# Autodesk Inventor assembly: 前後直動
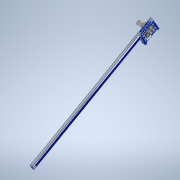
[picture p0: Inventor's stored thumbnail of the model, 180x180]
Saved by Autodesk Inventor 2020.3 (Build 243373000, 373)
## iProperties
Created: 2020-07-05
Part Number: 前後直動
Document SubType Name: Assembly
Designer: totot
Mass: 657.606 g
Surface Area: 2611.22 cm^2
Volume: 274.849 cm^3
Density: 2.39261 g/cm^3
Author: totot
## Documents named in this file (10)
- D:\mysvn\ロボコン\キャチロボ\キャチロボ設計図\ロボット\ハンド\前後直動.iam
- D:\mysvn\ロボコン\キャチロボ\キャチロボ設計図\ロボット\ハンド\12ｘ12_1.ipt
- D:\mysvn\ロボコン\キャチロボ\キャチロボ設計図\ロボット\共有パーツ\DR1-2000_On2.ipt
- D:\mysvn\ロボコン\キャチロボ\キャチロボ設計図\ロボット\ハンド\前後直動12x12_2.ipt
- D:\mysvn\ロボコン\キャチロボ\キャチロボ設計図\ロボット\ハンド\前後直動12x12_3.ipt
- D:\mysvn\ロボコン\キャチロボ\キャチロボ設計図\ロボット\ハンド\前後直動12x12_4.ipt
- D:\mysvn\ロボコン\キャチロボ\キャチロボ設計図\ロボット\共有パーツ\RS_380.ipt
- D:\mysvn\ロボコン\キャチロボ\キャチロボ設計図\ロボット\ハンド\前後直動9x9x24.ipt
- D:\mysvn\ロボコン\キャチロボ\キャチロボ設計図\ロボット\共有パーツ\ポテンションメーター_BI-7284.ipt
- D:\mysvn\ロボコン\キャチロボ\キャチロボ設計図\ロボット\共有パーツ\PS1-20_On.ipt
## Components (14 placed, 9 different names)
1. 12ｘ12_1:1 — メイト:1, フラッシュ:1, フラッシュ:2, 挿入:17, 挿入:18, 挿入:19, 挿入:20, 挿入:21, 挿入:26, 挿入:31, 挿入:32, 挿入:34, 挿入:35
2. DR1-2000_On2:1 — メイト:1, フラッシュ:1, フラッシュ:2
3. 前後直動t5_1 — 挿入:15, 挿入:16, 挿入:20, 挿入:21, 挿入:22, 挿入:23, 正接:1, メイト:2
4. RS_380:1 — 挿入:15, 挿入:16
5. 12ｘ12_1:2 — 挿入:17, 挿入:18, 挿入:19
6. 前後直動12x12_3:1 — 挿入:22, 挿入:23, 挿入:24, 挿入:25, 挿入:27, 挿入:30
7. 前後直動12x12_2:1 — 挿入:24, 挿入:28, 挿入:31, 挿入:36
8. 前後直動12x12_2:2 — 挿入:25, 挿入:26, 挿入:29, 挿入:32, 挿入:33
9. 前後直動9x9x24:1 — 挿入:27, 挿入:29
10. 前後直動9x9x24:2 — 挿入:28, 挿入:30
11. 前後直動9x9x24:3 — 挿入:33, 挿入:34
12. 前後直動9x9x24:4 — 挿入:35, 挿入:36
13. ポテンションメーター_BI-7284:1 — 正接:1, メイト:2, 正接:2, メイト:3
14. PS1-20_On:1 — 正接:2, メイト:3
## Relationships (29: Insert 22, Mate 3, Flush 2, Tangent 2)
- メイト:1 [Mate]: 12ｘ12_1:1 ↔ DR1-2000_On2:1
- フラッシュ:1 [Flush] (20 mm): 12ｘ12_1:1 ↔ DR1-2000_On2:1
- フラッシュ:2 [Flush] (-6 mm): 12ｘ12_1:1 ↔ DR1-2000_On2:1
- 挿入:15 [Insert]: 前後直動t5_1 ↔ RS_380:1
- 挿入:16 [Insert]: 前後直動t5_1 ↔ RS_380:1
- 挿入:17 [Insert]: 12ｘ12_1:1 ↔ 12ｘ12_1:2
- 挿入:18 [Insert]: 12ｘ12_1:1 ↔ 12ｘ12_1:2
- 挿入:19 [Insert]: 12ｘ12_1:1 ↔ 12ｘ12_1:2
- 挿入:20 [Insert]: 12ｘ12_1:1 ↔ 前後直動t5_1
- 挿入:21 [Insert]: 12ｘ12_1:1 ↔ 前後直動t5_1
- 挿入:22 [Insert]: 前後直動t5_1 ↔ 前後直動12x12_3:1
- 挿入:23 [Insert]: 前後直動t5_1 ↔ 前後直動12x12_3:1
- 挿入:24 [Insert]: 前後直動12x12_3:1 ↔ 前後直動12x12_2:1
- 挿入:25 [Insert]: 前後直動12x12_3:1 ↔ 前後直動12x12_2:2
- 挿入:26 [Insert]: 12ｘ12_1:1 ↔ 前後直動12x12_2:2
- 挿入:27 [Insert]: 前後直動12x12_3:1 ↔ 前後直動9x9x24:1
- 挿入:28 [Insert]: 前後直動12x12_2:1 ↔ 前後直動9x9x24:2
- 挿入:29 [Insert]: 前後直動12x12_2:2 ↔ 前後直動9x9x24:1
- 挿入:30 [Insert]: 前後直動12x12_3:1 ↔ 前後直動9x9x24:2
- 挿入:31 [Insert]: 12ｘ12_1:1 ↔ 前後直動12x12_2:1
- 挿入:32 [Insert]: 12ｘ12_1:1 ↔ 前後直動12x12_2:2
- 挿入:33 [Insert]: 前後直動12x12_2:2 ↔ 前後直動9x9x24:3
- 挿入:34 [Insert]: 12ｘ12_1:1 ↔ 前後直動9x9x24:3
- 挿入:35 [Insert]: 12ｘ12_1:1 ↔ 前後直動9x9x24:4
- 挿入:36 [Insert]: 前後直動12x12_2:1 ↔ 前後直動9x9x24:4
- 正接:1 [Tangent]: 前後直動t5_1 ↔ ポテンションメーター_BI-7284:1
- メイト:2 [Mate]: 前後直動t5_1 ↔ ポテンションメーター_BI-7284:1
- 正接:2 [Tangent]: ポテンションメーター_BI-7284:1 ↔ PS1-20_On:1
- メイト:3 [Mate]: ポテンションメーター_BI-7284:1 ↔ PS1-20_On:1
